# Autodesk Inventor assembly: main gripper assembly
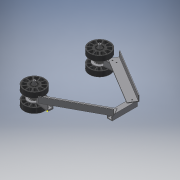
[picture p0: Inventor's stored thumbnail of the model, 180x180]
Saved by Autodesk Inventor 2018 (Build 220112000, 112)
## iProperties
Created: 2019-02-23
Part Number: main gripper assembly
Document SubType Name: Assembly
Designer: s-2513225
Author: s-2513225
## Documents named in this file (8)
- C:\Users\Tiberus\Documents\GitHub\2019CAD\NEW NEW GRIPPER (feb 23)\main gripper assembly.iam
- C:\Users\Tiberus\Documents\GitHub\2019CAD\NEW NEW GRIPPER (feb 23)\wheel tip connector 1.ipt
- C:\Users\Tiberus\Documents\GitHub\2019CAD\NEW NEW GRIPPER (feb 23)\angle iron with  holes 2.ipt
- C:\Users\Tiberus\Documents\GitHub\2019CAD\NEW NEW GRIPPER (feb 23)\base mount.ipt
- C:\Users\Tiberus\Documents\GitHub\2019CAD\NEW NEW GRIPPER (feb 23)\wheel tip assembly 2018 ver.iam
- C:\Users\Tiberus\Documents\GitHub\2019CAD\NEW NEW GRIPPER (feb 23)\wheel tip connector 1_MIR.ipt
- C:\Users\Tiberus\Documents\GitHub\2019CAD\NEW NEW GRIPPER (feb 23)\angle iron with  holes 2_MIR.ipt
- C:\Users\Tiberus\Documents\GitHub\2019CAD\NEW NEW GRIPPER (feb 23)\wheel tip assembly 2018 ver_MIR.iam
## Components (7 placed, 7 different names)
1. wheel tip connector 1:1 — Mate:12, Mate:23, Mate:25
2. angle iron with  holes 2:1 — Mate:12, Mate:14, Mate:19, Mate:20, Mate:21, Mate:24
3. base mount:1 — Mate:14, Mate:19, Mate:26, Mate:27, Mate:34, Mate:35
4. wheel tip assembly 2018 ver:1 [sub-assembly] — Mate:20, Mate:21, Mate:23, Mate:24, Mate:25
5. wheel tip connector 1_MIR:1 — Mate:28, Mate:29, Mate:31
6. angle iron with  holes 2_MIR:1 — Mate:28, Mate:30, Mate:32, Mate:33, Mate:34, Mate:35
7. wheel tip assembly 2018 ver_MIR:1 [sub-assembly] — Mate:29, Mate:30, Mate:31, Mate:32, Mate:33
## Relationships (19: Mate 18, Flush 1)
- Mate:12: wheel tip connector 1:1 ↔ angle iron with  holes 2:1
- Mate:14: angle iron with  holes 2:1 ↔ base mount:1
- Mate:19: angle iron with  holes 2:1 ↔ base mount:1
- Mate:20: angle iron with  holes 2:1 ↔ wheel tip assembly 2018 ver:1
- Mate:21: angle iron with  holes 2:1 ↔ wheel tip assembly 2018 ver:1
- Mate:23: wheel tip connector 1:1 ↔ wheel tip assembly 2018 ver:1
- Mate:24: angle iron with  holes 2:1 ↔ wheel tip assembly 2018 ver:1
- Mate:25: wheel tip connector 1:1 ↔ wheel tip assembly 2018 ver:1
- Mate:26: base mount:1
- Mate:27: base mount:1
- Flush:1 (63.5 mm)
- Mate:28: wheel tip connector 1_MIR:1 ↔ angle iron with  holes 2_MIR:1
- Mate:29: wheel tip connector 1_MIR:1 ↔ wheel tip assembly 2018 ver_MIR:1
- Mate:30: angle iron with  holes 2_MIR:1 ↔ wheel tip assembly 2018 ver_MIR:1
- Mate:31: wheel tip connector 1_MIR:1 ↔ wheel tip assembly 2018 ver_MIR:1
- Mate:32: angle iron with  holes 2_MIR:1 ↔ wheel tip assembly 2018 ver_MIR:1
- Mate:33: angle iron with  holes 2_MIR:1 ↔ wheel tip assembly 2018 ver_MIR:1
- Mate:34: base mount:1 ↔ angle iron with  holes 2_MIR:1
- Mate:35: base mount:1 ↔ angle iron with  holes 2_MIR:1
